# Autodesk Inventor assembly: b5
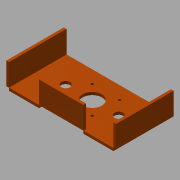
[picture p0: Inventor's stored thumbnail of the model, 180x180]
Saved by Autodesk Inventor 2016 (Build 200138000, 138)
## iProperties
Created: 2016-06-11
Part Number: b5
Document SubType Name: Assembly
Designer: daniel
Author: daniel
## Documents named in this file (4)
- C:\Users\daniel\Documents\GitHub\cardboard-stage-metric\stage\b5.iam
- C:\Users\daniel\Documents\GitHub\cardboard-stage-metric\stage\b3b.ipt
- C:\Users\daniel\Documents\GitHub\cardboard-stage-metric\stage\b3c.ipt
- C:\Users\daniel\Documents\GitHub\cardboard-stage-metric\stage\b5a.ipt
## Components (4 placed, 3 different names)
1. b5a:1 — Mate:2, Mate:4, Mate:7, Mate:8, Mate:9, Mate:10, Mate:11, Flush:1, Flush:2
2. b3b:1 — Mate:4, Mate:11, Flush:2
3. b3c:1 — Mate:2, Mate:8, Mate:9
4. b3b:2 — Mate:7, Mate:10, Flush:1
## Relationships (9: Mate 7, Flush 2)
- Mate:2: b5a:1 ↔ b3c:1
- Mate:4: b5a:1 ↔ b3b:1
- Mate:7: b5a:1 ↔ b3b:2
- Mate:8: b5a:1 ↔ b3c:1
- Mate:9: b5a:1 ↔ b3c:1
- Mate:10: b5a:1 ↔ b3b:2
- Mate:11: b5a:1 ↔ b3b:1
- Flush:1: b5a:1 ↔ b3b:2
- Flush:2: b5a:1 ↔ b3b:1
